# Autodesk Inventor assembly: Environment
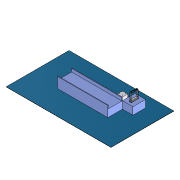
[picture p0: Inventor's stored thumbnail of the model, 180x180]
Saved by Autodesk Inventor 2021 (Build 250183000, 183)
## iProperties
Created: 2021-04-02
Part Number: Environment
Document SubType Name: Assembly
Designer: Tran Duc Viet
Mass: 898328 g
Surface Area: 394070 cm^2
Volume: 898328 cm^3
Density: 1 g/cm^3
Author: Tran Duc Viet
## Documents named in this file (3)
- C:\Users\davei\Desktop\School\Léto 2020-2021\VRM\Projects\P2\Environment.iam
- C:\Users\davei\Desktop\School\Léto 2020-2021\VRM\Projects\P2\Environment.ipt
- C:\Users\davei\Desktop\School\Léto 2020-2021\VRM\Projects\P2\Box.ipt
## Components (2 placed, 2 different names)
1. Environment:1 — Mate:1, Mate:2, Flush:1, Flush:2
2. Box:1 — Mate:2, Flush:1, Flush:2
## Relationships (4: Mate 2, Flush 2)
- Mate:1: Environment:1
- Mate:2: Environment:1 ↔ Box:1
- Flush:1 (125 mm): Environment:1 ↔ Box:1
- Flush:2 (-200 mm): Environment:1 ↔ Box:1
